# Autodesk Inventor assembly: Center Frame SEC
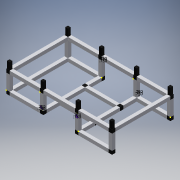
[picture p0: Inventor's stored thumbnail of the model, 180x180]
Saved by Autodesk Inventor 2017 (Build 210142000, 142)
## iProperties
Created: 2019-12-06
Part Number: Center Frame SEC
Document SubType Name: Assembly
Designer: S346553810
Author: S346553810
## Documents named in this file (7)
- \\ad.ocdsb.ca\studenthome\3\S338674153\FRC 2020\FullRobotRefactor\SubFrame\Center Frame SEC.iam
- \\ad.ocdsb.ca\studenthome\3\S338674153\FRC 2020\FullRobotRefactor\SubFrame\Center Assembly.iam
- \\ad.ocdsb.ca\studenthome\3\S338674153\FRC 2020\FullRobotRefactor\SubFrame\Frame End.iam
- \\ad.ocdsb.ca\studenthome\3\S338674153\FRC 2020\FullRobotRefactor\SubFrame\90 joint piece.ipt
- \\ad.ocdsb.ca\studenthome\3\S338674153\FRC 2020\FullRobotRefactor\SubFrame\Kipp K0619.ipt
- \\ad.ocdsb.ca\studenthome\3\S338674153\FRC 2020\FullRobotRefactor\SubFrame\lower piece.ipt
- \\ad.ocdsb.ca\studenthome\3\S338674153\FRC 2020\FullRobotRefactor\SubFrame\roller hole piece.ipt
## Components (12 placed, 6 different names)
1. Center Assembly:1 [sub-assembly] — Flush:2, Mate:12, Flush:9, Mate:13, Mate:26, Flush:22, Flush:23
2. Frame End:1 [sub-assembly] — Flush:4, Mate:7, Mate:8, Mate:9, Mate:12, Flush:9, Mate:13, Mate:18, Flush:12, Flush:13, Flush:14, Flush:15, Mate:20
3. Frame End:2 [sub-assembly] — Flush:2, Mate:14, Flush:10, Mate:15, Mate:16, Mate:17, Flush:11, Mate:25, Mate:26, Flush:22, Flush:23
4. 90 joint piece:1 — Mate:24, Flush:20, Flush:21, Mate:25
5. 90 joint piece:2 — Mate:23, Flush:18, Flush:19
6. Kipp K0619:1 — Flush:4, Mate:7, Mate:8, Mate:10, Flush:8, Mate:19
7. Kipp K0619:2 — Mate:9, Mate:11, Mate:20, Mate:27
8. lower piece:1 — Mate:10, Flush:8, Mate:11, Mate:27
9. roller hole piece:2 — Mate:16, Mate:17, Flush:11, Mate:23, Flush:18, Flush:19
10. roller hole piece:3 — Mate:14, Flush:10, Mate:15, Mate:24, Flush:20, Flush:21
11. roller hole piece:4 — Flush:14, Flush:15, Mate:19
12. roller hole piece:5 — Mate:18, Flush:12, Flush:13
## Relationships (35: Mate 19, Flush 16)
- Flush:2: Center Assembly:1 ↔ Frame End:2
- Flush:4: Frame End:1 ↔ Kipp K0619:1
- Mate:7: Frame End:1 ↔ Kipp K0619:1
- Mate:8: Frame End:1 ↔ Kipp K0619:1
- Mate:9: Frame End:1 ↔ Kipp K0619:2
- Mate:10: Kipp K0619:1 ↔ lower piece:1
- Flush:8: Kipp K0619:1 ↔ lower piece:1
- Mate:11: Kipp K0619:2 ↔ lower piece:1
- Mate:12: Center Assembly:1 ↔ Frame End:1
- Flush:9: Center Assembly:1 ↔ Frame End:1
- Mate:13: Center Assembly:1 ↔ Frame End:1
- Mate:14: Frame End:2 ↔ roller hole piece:3
- Flush:10: Frame End:2 ↔ roller hole piece:3
- Mate:15: Frame End:2 ↔ roller hole piece:3
- Mate:16: Frame End:2 ↔ roller hole piece:2
- Mate:17: Frame End:2 ↔ roller hole piece:2
- Flush:11: Frame End:2 ↔ roller hole piece:2
- Mate:18: Frame End:1 ↔ roller hole piece:5
- Flush:12: Frame End:1 ↔ roller hole piece:5
- Flush:13: Frame End:1 ↔ roller hole piece:5
- Flush:14: Frame End:1 ↔ roller hole piece:4
- Flush:15: Frame End:1 ↔ roller hole piece:4
- Mate:19: Kipp K0619:1 ↔ roller hole piece:4
- Mate:20: Frame End:1 ↔ Kipp K0619:2
- Mate:23: 90 joint piece:2 ↔ roller hole piece:2
- Flush:18: 90 joint piece:2 ↔ roller hole piece:2
- Flush:19: 90 joint piece:2 ↔ roller hole piece:2
- Mate:24: 90 joint piece:1 ↔ roller hole piece:3
- Flush:20: 90 joint piece:1 ↔ roller hole piece:3
- Flush:21: 90 joint piece:1 ↔ roller hole piece:3
- Mate:25: Frame End:2 ↔ 90 joint piece:1
- Mate:26: Center Assembly:1 ↔ Frame End:2
- Flush:22: Center Assembly:1 ↔ Frame End:2
- Flush:23: Center Assembly:1 ↔ Frame End:2
- Mate:27: Kipp K0619:2 ↔ lower piece:1
